# Autodesk Inventor assembly: printer2
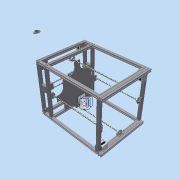
[picture p0: Inventor's stored thumbnail of the model, 180x180]
Saved by Autodesk Inventor 2015 (Build 190159000, 159)
## iProperties
Created: 2016-06-24
Part Number: printer2
Document SubType Name: Assembly
Designer: Dustin
Author: Dustin
## Documents named in this file (20)
- E:\Documents\3D Printer\Parts\New Printer\printer2.iam
- E:\Documents\3D Printer\Parts\New Printer\20x20x9in.ipt
- E:\Documents\3D Printer\Parts\New Printer\20x20x27cm.ipt
- E:\Documents\3D Printer\Parts\New Printer\20x20x3in.ipt
- E:\Documents\3D Printer\Parts\New Printer\heated bed.ipt
- E:\Documents\3D Printer\Parts\New Printer\NEMA17.ipt
- E:\Documents\3D Printer\Parts\New Printer\.375 - 8 (4 start) acme thread.ipt
- E:\Documents\3D Printer\Parts\New Printer\leadscrew corners.ipt
- E:\Documents\3D Printer\Parts\New Printer\bed plate.ipt
- E:\Documents\3D Printer\Parts\New Printer\Imported Components\GT2_20teeth_pulley\GT2_20teeth_pulley.ipt
- E:\Documents\3D Printer\Parts\New Printer\6mm_rod_265.ipt
- E:\Documents\3D Printer\Parts\New Printer\motor mount.ipt
- E:\Documents\3D Printer\Parts\New Printer\20x20x5cm.ipt
- E:\Documents\3D Printer\Parts\New Printer\extruder.iam
- E:\Documents\3D Printer\Parts\New Printer\X smooth mount.ipt
- E:\Documents\3D Printer\Parts\New Printer\m3x20.ipt
- E:\Documents\3D Printer\Parts\New Printer\Corner mount.ipt
- E:\Documents\3D Printer\Parts\New Printer\m4 bearing assembly.iam
- E:\Documents\3D Printer\Parts\New Printer\m4 bearing assembly 30mm.iam
- E:\Documents\3D Printer\Parts\New Printer\KFL08.iam
## Components (83 placed, 19 different names)
1. 20x20x9in:1 — Mate:2, Flush:3, Flush:4, Flush:7
2. 20x20x9in:2 — Mate:4, Flush:8, Flush:9, Mate:6, Mate:39, Mate:52, Flush:53, Flush:64, Mate:66
3. 20x20x9in:3 — Mate:5, Flush:10, Flush:11, Flush:12, Flush:13, Mate:48, Flush:51, Mate:59, Flush:65, Mate:67
4. 20x20x9in:4 — Mate:1, Flush:1, Flush:2, Mate:3, Flush:5, Flush:6
5. 20x20x27cm:1 — Mate:1, Flush:1, Flush:2, Mate:2, Flush:3, Flush:4, Mate:38, Flush:40, Flush:41
6. 20x20x27cm:2 — Mate:3, Flush:5, Flush:6, Flush:7
7. 20x20x27cm:3 — Mate:4, Flush:8, Flush:9, Mate:5, Flush:10, Flush:11, Mate:11, Mate:12, Flush:24, Flush:25, Flush:26, Flush:27, Mate:50, Mate:60, Flush:60, Flush:61, Mate:65, Mate:85
8. 20x20x27cm:4 — Mate:6, Flush:12, Flush:13, Mate:10, Mate:13, Flush:21, Flush:22, Flush:23, Flush:28, Flush:29, Mate:54, Flush:54, Flush:62, Mate:61, Flush:63, Mate:68
9. 20x20x27cm:5 — Mate:13, Flush:21, Flush:28, Flush:29
10. 20x20x27cm:6 — Mate:12, Flush:26, Flush:27, Mate:14, Flush:30, Flush:31
11. 20x20x27cm:7 — Mate:11, Flush:24, Flush:25
12. 20x20x27cm:8 — Mate:10, Flush:22, Flush:23
13. 20x20x3in:1 — Mate:37, Flush:32, Flush:33
14. 20x20x3in:2 — Mate:36, Flush:38, Flush:39, Mate:38, Flush:40, Flush:41
15. 20x20x3in:3 — Mate:34, Flush:36, Flush:37
16. 20x20x3in:4 — Mate:35, Flush:34, Flush:35
17. 20x20x9in:5 — Mate:40, Flush:47, Flush:48, Flush:73, Flush:105
18. 20x20x9in:6 — Mate:44, Flush:50, Flush:77, Mate:83, Flush:104
19. 20x20x27cm:9 — Mate:14, Flush:30, Flush:31, Mate:34, Mate:37, Flush:32, Flush:33, Flush:38, Flush:39, Mate:42, Flush:49, Mate:74, Mate:75, Flush:74, Flush:75, Flush:76, Angle:3
20. 20x20x27cm:10 — Mate:35, Mate:36, Flush:34, Flush:35, Flush:36, Flush:37, Mate:46, Flush:71, Flush:72, Mate:72, Mate:73, Flush:78
21. heated bed:1 — Mate:58, Tangent:5, Tangent:6
22. NEMA17:1 — Mate:39, Flush:64, Insert:7, Mate:85, Insert:25, Insert:26
23. NEMA17:2 — Mate:59, Flush:65, Insert:6, Insert:20, Insert:21
24. .375 - 8 (4 start) acme thread:1 — Tangent:1, Flush:58, Insert:3, Tangent:18, Tangent:24, Tangent:56
25. .375 - 8 (4 start) acme thread:2 — Tangent:4, Flush:57, Insert:1, Tangent:20, Tangent:25, Tangent:54
26. .375 - 8 (4 start) acme thread:3 — Tangent:3, Flush:56, Insert:5, Tangent:14
27. .375 - 8 (4 start) acme thread:4 — Tangent:2, Flush:55, Insert:4, Tangent:16, Tangent:21, Tangent:53
28. leadscrew corners:1 — Mate:40, Flush:47, Tangent:1, Mate:57, Tangent:57, Flush:111
29. leadscrew corners:2 — Mate:42, Flush:48, Tangent:4, Mate:80, Flush:110, Tangent:55
30. leadscrew corners:3 — Mate:44, Flush:49, Tangent:3
31. leadscrew corners:4 — Mate:46, Flush:50, Tangent:2, Flush:109
32. leadscrew corners:5 — Mate:48, Flush:51, Flush:58, Tangent:18, Mate:67
33. leadscrew corners:6 — Mate:50, Flush:57, Tangent:20, Mate:65
34. leadscrew corners:7 — Mate:54, Flush:54, Flush:55, Tangent:16, Mate:68
35. leadscrew corners:8 — Mate:52, Flush:53, Flush:56, Tangent:14, Mate:66
36. bed plate:1 — Mate:57, Mate:58, Tangent:5, Tangent:6, Mate:80, Tangent:21, Tangent:24, Tangent:25, Angle:3
37. GT2_20teeth_pulley:1 — Insert:1
38. GT2_20teeth_pulley:2 — Insert:5
39. GT2_20teeth_pulley:3 — Insert:3
40. GT2_20teeth_pulley:4 — Insert:4
41. 20x20x27cm:11 — Mate:60, Flush:60, Flush:61
42. 20x20x27cm:12 — Flush:62, Mate:61, Flush:63
43. GT2_20teeth_pulley:5 — Insert:6
44. GT2_20teeth_pulley:6 — Insert:7
45. 6mm_rod_265:1 — Flush:68, Mate:83, Angle:1, Tangent:22, Insert:28, Tangent:47, Insert:33, Tangent:51, Angle:26, Angle:27
46. 6mm_rod_265:2 — Flush:68, Tangent:23, Insert:27, Tangent:48, Angle:25, Tangent:52
47. NEMA17:3 — Insert:18, Insert:19, Mate:87, Mate:88, Insert:32
48. NEMA17:4 — Insert:23, Insert:24, Mate:90, Tangent:34, Insert:31, Mate:98
49. motor mount:1 — Insert:18, Insert:19, Mate:86
50. 20x20x5cm:1 — Flush:71, Flush:72, Mate:72
51. 20x20x5cm:2 — Mate:75, Flush:73, Flush:74
52. 20x20x5cm:3 — Mate:74, Flush:75, Flush:76, Flush:79, Flush:80, Mate:76
53. 20x20x5cm:4 — Mate:73, Flush:77, Flush:78, Mate:77, Flush:81, Flush:82
54. 20x20x27cm:13 — Mate:77, Flush:81, Flush:82, Mate:88, Mate:90
55. 20x20x27cm:14 — Flush:79, Flush:80, Mate:76, Mate:78, Flush:83, Flush:84, Mate:79, Flush:85, Flush:86, Flush:89, Mate:100, Flush:92
56. 20x20x9in:7 — Mate:78, Flush:83, Flush:84, Angle:2, Mate:84, Mate:89, Mate:98, Flush:91, Mate:101, Flush:106
57. 20x20x9in:8 — Mate:79, Flush:85, Flush:86, Mate:86, Mate:87, Flush:90
58. motor mount:2 — Insert:20, Insert:21
59. GT2_20teeth_pulley:7 — Insert:32
60. motor mount:3 — Insert:23, Insert:24, Mate:89
61. extruder:1 [sub-assembly] — Angle:1, Angle:2, Tangent:22, Tangent:23, Mate:84, Tangent:35, Angle:11, Mate:99, Tangent:36, Angle:12, Mate:102, Angle:21, Tangent:45, Angle:22, Tangent:46, Flush:100, Flush:101, Flush:106, Flush:107, Angle:27, Flush:108
62. motor mount:4 — Insert:25, Insert:26
63. X smooth mount:1 — Insert:27, Insert:28, Angle:13, Tangent:37, Flush:93, Angle:16, Tangent:40, Flush:95, Tangent:51, Angle:25, Flush:104, Tangent:52
64. GT2_20teeth_pulley:8 — Tangent:34, Insert:31
65. m3x20:1 — Tangent:35, Angle:11, Mate:99, Flush:107
66. Corner mount:1 — Flush:89, Mate:100, Flush:90, Angle:19, Flush:98, Tangent:43, Angle:20, Tangent:44, Flush:99
67. Corner mount:2 — Flush:91, Mate:101, Flush:92, Angle:14, Tangent:38, Flush:94, Angle:15, Tangent:39, Mate:103
68. m3x20:2 — Tangent:36, Angle:12, Mate:102, Flush:108
69. m4 bearing assembly:1 [sub-assembly] — Angle:13, Tangent:37, Flush:93
70. m4 bearing assembly:2 [sub-assembly] — Angle:14, Tangent:38, Flush:94
71. m4 bearing assembly 30mm:1 [sub-assembly] — Angle:15, Tangent:39, Mate:103
72. m4 bearing assembly 30mm:2 [sub-assembly] — Angle:16, Tangent:40, Flush:95
73. m4 bearing assembly:3 [sub-assembly] — Tangent:50, Angle:24, Flush:103
74. m4 bearing assembly 30mm:3 [sub-assembly] — Tangent:49, Angle:23, Flush:102
75. m4 bearing assembly:4 [sub-assembly] — Angle:19, Flush:98, Tangent:43
76. m4 bearing assembly 30mm:4 [sub-assembly] — Angle:20, Tangent:44, Flush:99
77. m3x20:3 — Angle:21, Tangent:45, Flush:100
78. m3x20:4 — Angle:22, Tangent:46, Flush:101
79. X smooth mount:2 — Tangent:47, Tangent:48, Insert:33, Tangent:49, Tangent:50, Angle:23, Angle:24, Flush:102, Flush:103, Angle:26, Flush:105
80. KFL08:1 [sub-assembly] — Flush:109, Tangent:53
81. KFL08:2 [sub-assembly] — Flush:110, Tangent:54, Tangent:55
82. KFL08:3 [sub-assembly]
83. KFL08:4 [sub-assembly] — Tangent:56, Tangent:57, Flush:111
## Relationships (230: Flush 96, Mate 60, Tangent 37, Insert 19, Angle 18)
- Mate:1: 20x20x9in:4 ↔ 20x20x27cm:1
- Flush:1: 20x20x9in:4 ↔ 20x20x27cm:1
- Flush:2: 20x20x9in:4 ↔ 20x20x27cm:1
- Mate:2: 20x20x9in:1 ↔ 20x20x27cm:1
- Flush:3: 20x20x9in:1 ↔ 20x20x27cm:1
- Flush:4: 20x20x9in:1 ↔ 20x20x27cm:1
- Mate:3: 20x20x9in:4 ↔ 20x20x27cm:2
- Flush:5: 20x20x9in:4 ↔ 20x20x27cm:2
- Flush:6: 20x20x9in:4 ↔ 20x20x27cm:2
- Flush:7: 20x20x9in:1 ↔ 20x20x27cm:2
- Mate:4: 20x20x9in:2 ↔ 20x20x27cm:3
- Flush:8: 20x20x9in:2 ↔ 20x20x27cm:3
- Flush:9: 20x20x9in:2 ↔ 20x20x27cm:3
- Mate:5: 20x20x9in:3 ↔ 20x20x27cm:3
- Flush:10: 20x20x9in:3 ↔ 20x20x27cm:3
- Flush:11: 20x20x9in:3 ↔ 20x20x27cm:3
- Mate:6: 20x20x9in:2 ↔ 20x20x27cm:4
- Flush:12: 20x20x9in:3 ↔ 20x20x27cm:4
- Flush:13: 20x20x9in:3 ↔ 20x20x27cm:4
- [Mate]: 20x20x9in:6 ↔ 20x20x27cm:9
- [Flush]: 20x20x9in:6 ↔ 20x20x27cm:9
- [Flush]: 20x20x9in:6 ↔ 20x20x27cm:9
- [Mate]: 20x20x9in:5 ↔ 20x20x27cm:9
- [Flush]: 20x20x9in:5 ↔ 20x20x27cm:9
- [Flush]: 20x20x9in:5 ↔ 20x20x27cm:9
- [Mate]: 20x20x9in:6 ↔ 20x20x27cm:10
- [Flush]: 20x20x9in:6 ↔ 20x20x27cm:10
- [Flush]: 20x20x9in:6 ↔ 20x20x27cm:10
- [Flush]: 20x20x9in:5 ↔ 20x20x27cm:10
- Mate:10: 20x20x27cm:4 ↔ 20x20x27cm:8
- Mate:11: 20x20x27cm:3 ↔ 20x20x27cm:7
- Mate:12: 20x20x27cm:3 ↔ 20x20x27cm:6
- Mate:13: 20x20x27cm:4 ↔ 20x20x27cm:5
- Flush:21: 20x20x27cm:4 ↔ 20x20x27cm:5
- Flush:22: 20x20x27cm:4 ↔ 20x20x27cm:8
- Flush:23: 20x20x27cm:4 ↔ 20x20x27cm:8
- Flush:24: 20x20x27cm:3 ↔ 20x20x27cm:7
- Flush:25: 20x20x27cm:3 ↔ 20x20x27cm:7
- Flush:26: 20x20x27cm:3 ↔ 20x20x27cm:6
- Flush:27: 20x20x27cm:3 ↔ 20x20x27cm:6
- Flush:28: 20x20x27cm:4 ↔ 20x20x27cm:5
- Flush:29: 20x20x27cm:4 ↔ 20x20x27cm:5
- Mate:14: 20x20x27cm:6 ↔ 20x20x27cm:9
- Flush:30: 20x20x27cm:6 ↔ 20x20x27cm:9
- Flush:31: 20x20x27cm:6 ↔ 20x20x27cm:9
- Mate:35: 20x20x3in:4 ↔ 20x20x27cm:10
- Mate:34: 20x20x3in:3 ↔ 20x20x27cm:9
- Mate:36: 20x20x3in:2 ↔ 20x20x27cm:10
- Mate:37: 20x20x3in:1 ↔ 20x20x27cm:9
- Flush:32: 20x20x3in:1 ↔ 20x20x27cm:9
- Flush:33: 20x20x3in:1 ↔ 20x20x27cm:9
- Flush:34: 20x20x3in:4 ↔ 20x20x27cm:10
- Flush:35: 20x20x3in:4 ↔ 20x20x27cm:10
- Flush:36: 20x20x3in:3 ↔ 20x20x27cm:10
- Flush:37: 20x20x3in:3 ↔ 20x20x27cm:10
- Flush:38: 20x20x3in:2 ↔ 20x20x27cm:9
- Flush:39: 20x20x3in:2 ↔ 20x20x27cm:9
- Mate:38: 20x20x27cm:1 ↔ 20x20x3in:2
- Flush:40: 20x20x27cm:1 ↔ 20x20x3in:2
- Flush:41: 20x20x27cm:1 ↔ 20x20x3in:2
- Mate:39: 20x20x9in:2 ↔ NEMA17:1
- Mate:40: 20x20x9in:5 ↔ leadscrew corners:1
- Flush:47: 20x20x9in:5 ↔ leadscrew corners:1
- Tangent:1: .375 - 8 (4 start) acme thread:1 ↔ leadscrew corners:1
- Mate:42: 20x20x27cm:9 ↔ leadscrew corners:2
- Flush:48: 20x20x9in:5 ↔ leadscrew corners:2
- Mate:44: 20x20x9in:6 ↔ leadscrew corners:3
- Flush:49: 20x20x27cm:9 ↔ leadscrew corners:3
- Mate:46: 20x20x27cm:10 ↔ leadscrew corners:4
- Flush:50: 20x20x9in:6 ↔ leadscrew corners:4
- Tangent:2: .375 - 8 (4 start) acme thread:4 ↔ leadscrew corners:4
- Tangent:3: .375 - 8 (4 start) acme thread:3 ↔ leadscrew corners:3
- Tangent:4: .375 - 8 (4 start) acme thread:2 ↔ leadscrew corners:2
- Mate:48: 20x20x9in:3 ↔ leadscrew corners:5
- Flush:51: 20x20x9in:3 ↔ leadscrew corners:5
- Mate:50: 20x20x27cm:3 ↔ leadscrew corners:6
- Mate:52: 20x20x9in:2 ↔ leadscrew corners:8
- Flush:53: 20x20x9in:2 ↔ leadscrew corners:8
- Mate:54: 20x20x27cm:4 ↔ leadscrew corners:7
- Flush:54: 20x20x27cm:4 ↔ leadscrew corners:7
- Flush:55 (5 mm): .375 - 8 (4 start) acme thread:4 ↔ leadscrew corners:7
- Flush:56 (5 mm): .375 - 8 (4 start) acme thread:3 ↔ leadscrew corners:8
- Flush:57 (5 mm): .375 - 8 (4 start) acme thread:2 ↔ leadscrew corners:6
- Flush:58 (5 mm): .375 - 8 (4 start) acme thread:1 ↔ leadscrew corners:5
- Mate:57: leadscrew corners:1 ↔ bed plate:1
- Mate:58 (6 mm): heated bed:1 ↔ bed plate:1
- Tangent:5: heated bed:1 ↔ bed plate:1
- Tangent:6: heated bed:1 ↔ bed plate:1
- Mate:59: 20x20x9in:3 ↔ NEMA17:2
- Insert:1 (-19.05 mm): .375 - 8 (4 start) acme thread:2 ↔ GT2_20teeth_pulley:1
- Insert:3 (-19.05 mm): .375 - 8 (4 start) acme thread:1 ↔ GT2_20teeth_pulley:3
- Insert:4 (-19.05 mm): .375 - 8 (4 start) acme thread:4 ↔ GT2_20teeth_pulley:4
- Insert:5 (-19.05 mm): .375 - 8 (4 start) acme thread:3 ↔ GT2_20teeth_pulley:2
- Mate:60: 20x20x27cm:3 ↔ 20x20x27cm:11
- Flush:60: 20x20x27cm:3 ↔ 20x20x27cm:11
- Flush:61: 20x20x27cm:3 ↔ 20x20x27cm:11
- Flush:62: 20x20x27cm:4 ↔ 20x20x27cm:12
- Mate:61: 20x20x27cm:4 ↔ 20x20x27cm:12
- Flush:63: 20x20x27cm:4 ↔ 20x20x27cm:12
- Flush:64: 20x20x9in:2 ↔ NEMA17:1
- Flush:65: 20x20x9in:3 ↔ NEMA17:2
- Insert:6 (-3.81 mm): NEMA17:2 ↔ GT2_20teeth_pulley:5
- Insert:7 (-3.81 mm): NEMA17:1 ↔ GT2_20teeth_pulley:6
- Flush:68: 6mm_rod_265:1 ↔ 6mm_rod_265:2
- Tangent:14: .375 - 8 (4 start) acme thread:3 ↔ leadscrew corners:8
- Tangent:16 (-1 mm): .375 - 8 (4 start) acme thread:4 ↔ leadscrew corners:7
- Tangent:18: .375 - 8 (4 start) acme thread:1 ↔ leadscrew corners:5
- Tangent:20 (-1 mm): .375 - 8 (4 start) acme thread:2 ↔ leadscrew corners:6
- Mate:65: 20x20x27cm:3 ↔ leadscrew corners:6
- Mate:66: 20x20x9in:2 ↔ leadscrew corners:8
- Mate:67: 20x20x9in:3 ↔ leadscrew corners:5
- Mate:68: 20x20x27cm:4 ↔ leadscrew corners:7
- Insert:18: NEMA17:3 ↔ motor mount:1
- Insert:19: NEMA17:3 ↔ motor mount:1
- Flush:71: 20x20x27cm:10 ↔ 20x20x5cm:1
- Flush:72: 20x20x27cm:10 ↔ 20x20x5cm:1
- Mate:72: 20x20x27cm:10 ↔ 20x20x5cm:1
- Mate:73: 20x20x27cm:10 ↔ 20x20x5cm:4
- Mate:74: 20x20x27cm:9 ↔ 20x20x5cm:3
- Mate:75: 20x20x27cm:9 ↔ 20x20x5cm:2
- Flush:73: 20x20x9in:5 ↔ 20x20x5cm:2
- Flush:74: 20x20x27cm:9 ↔ 20x20x5cm:2
- Flush:75: 20x20x27cm:9 ↔ 20x20x5cm:3
- Flush:76: 20x20x27cm:9 ↔ 20x20x5cm:3
- Flush:77: 20x20x9in:6 ↔ 20x20x5cm:4
- Flush:78: 20x20x27cm:10 ↔ 20x20x5cm:4
- Flush:79: 20x20x5cm:3 ↔ 20x20x27cm:14
- Flush:80: 20x20x5cm:3 ↔ 20x20x27cm:14
- Mate:76: 20x20x5cm:3 ↔ 20x20x27cm:14
- Mate:77: 20x20x5cm:4 ↔ 20x20x27cm:13
- Flush:81: 20x20x5cm:4 ↔ 20x20x27cm:13
- Flush:82: 20x20x5cm:4 ↔ 20x20x27cm:13
- Mate:78: 20x20x27cm:14 ↔ 20x20x9in:7
- Flush:83: 20x20x27cm:14 ↔ 20x20x9in:7
- Flush:84: 20x20x27cm:14 ↔ 20x20x9in:7
- Mate:79: 20x20x27cm:14 ↔ 20x20x9in:8
- Flush:85: 20x20x27cm:14 ↔ 20x20x9in:8
- Flush:86: 20x20x27cm:14 ↔ 20x20x9in:8
- Insert:20: NEMA17:2 ↔ motor mount:2
- Insert:21: NEMA17:2 ↔ motor mount:2
- Mate:80: leadscrew corners:2 ↔ bed plate:1
- Tangent:21: .375 - 8 (4 start) acme thread:4 ↔ bed plate:1
- Insert:23: NEMA17:4 ↔ motor mount:3
- Insert:24: NEMA17:4 ↔ motor mount:3
- Mate:83: 20x20x9in:6 ↔ 6mm_rod_265:1
- Angle:1 (0 deg): 6mm_rod_265:1 ↔ extruder:1
- Angle:2 (180 deg): 20x20x9in:7 ↔ extruder:1
- Tangent:22: 6mm_rod_265:1 ↔ extruder:1
- Tangent:23: 6mm_rod_265:2 ↔ extruder:1
- Mate:84 (25 mm): 20x20x9in:7 ↔ extruder:1
- Mate:85: 20x20x27cm:3 ↔ NEMA17:1
- Insert:25: NEMA17:1 ↔ motor mount:4
- Insert:26: NEMA17:1 ↔ motor mount:4
- Insert:27: 6mm_rod_265:2 ↔ X smooth mount:1
- Insert:28: 6mm_rod_265:1 ↔ X smooth mount:1
- Tangent:24: .375 - 8 (4 start) acme thread:1 ↔ bed plate:1
- Tangent:25: .375 - 8 (4 start) acme thread:2 ↔ bed plate:1
- Angle:3 (0 deg): 20x20x27cm:9 ↔ bed plate:1
- Mate:86: motor mount:1 ↔ 20x20x9in:8
- Mate:87: NEMA17:3 ↔ 20x20x9in:8
- Mate:88: NEMA17:3 ↔ 20x20x27cm:13
- Mate:89: 20x20x9in:7 ↔ motor mount:3
- Mate:90: NEMA17:4 ↔ 20x20x27cm:13
- Tangent:34: NEMA17:4 ↔ GT2_20teeth_pulley:8
- Insert:31 (5 mm): NEMA17:4 ↔ GT2_20teeth_pulley:8
- Mate:98: NEMA17:4 ↔ 20x20x9in:7
- Tangent:35: extruder:1 ↔ m3x20:1
- Angle:11 (180 deg): extruder:1 ↔ m3x20:1
- Mate:99 (14 mm): extruder:1 ↔ m3x20:1
- Flush:89: 20x20x27cm:14 ↔ Corner mount:1
- Mate:100: 20x20x27cm:14 ↔ Corner mount:1
- Flush:90: 20x20x9in:8 ↔ Corner mount:1
- Flush:91: 20x20x9in:7 ↔ Corner mount:2
- Mate:101: 20x20x9in:7 ↔ Corner mount:2
- Flush:92: 20x20x27cm:14 ↔ Corner mount:2
- Insert:32: NEMA17:3 ↔ GT2_20teeth_pulley:7
- Tangent:36: extruder:1 ↔ m3x20:2
- Angle:12 (180 deg): extruder:1 ↔ m3x20:2
- Mate:102 (10 mm): extruder:1 ↔ m3x20:2
- Angle:13 (180 deg): X smooth mount:1 ↔ m4 bearing assembly:1
- Tangent:37: X smooth mount:1 ↔ m4 bearing assembly:1
- Flush:93 (-5 mm): X smooth mount:1 ↔ m4 bearing assembly:1
- Angle:14 (0 deg): Corner mount:2 ↔ m4 bearing assembly:2
- Tangent:38: Corner mount:2 ↔ m4 bearing assembly:2
- Flush:94 (-6 mm): Corner mount:2 ↔ m4 bearing assembly:2
- Angle:15 (0 deg): Corner mount:2 ↔ m4 bearing assembly 30mm:1
- Tangent:39: Corner mount:2 ↔ m4 bearing assembly 30mm:1
- Mate:103 (15 mm): Corner mount:2 ↔ m4 bearing assembly 30mm:1
- Angle:16 (180 deg): X smooth mount:1 ↔ m4 bearing assembly 30mm:2
- Tangent:40: X smooth mount:1 ↔ m4 bearing assembly 30mm:2
- Flush:95: X smooth mount:1 ↔ m4 bearing assembly 30mm:2
- Angle:19 (0 deg): Corner mount:1 ↔ m4 bearing assembly:4
- Flush:98 (-6 mm): Corner mount:1 ↔ m4 bearing assembly:4
- Tangent:43: Corner mount:1 ↔ m4 bearing assembly:4
- Angle:20 (180 deg): Corner mount:1 ↔ m4 bearing assembly 30mm:4
- Tangent:44: Corner mount:1 ↔ m4 bearing assembly 30mm:4
- Flush:99 (1 mm): Corner mount:1 ↔ m4 bearing assembly 30mm:4
- Angle:21 (180 deg): extruder:1 ↔ m3x20:3
- Tangent:45: extruder:1 ↔ m3x20:3
- Angle:22 (180 deg): extruder:1 ↔ m3x20:4
- Tangent:46: extruder:1 ↔ m3x20:4
- Flush:100 (-6 mm): extruder:1 ↔ m3x20:3
- Flush:101 (-2 mm): extruder:1 ↔ m3x20:4
- Tangent:47: 6mm_rod_265:1 ↔ X smooth mount:2
- Tangent:48: 6mm_rod_265:2 ↔ X smooth mount:2
- Insert:33 (-20 mm): 6mm_rod_265:1 ↔ X smooth mount:2
- Tangent:49: m4 bearing assembly 30mm:3 ↔ X smooth mount:2
- Tangent:50: m4 bearing assembly:3 ↔ X smooth mount:2
- Angle:23 (180 deg): m4 bearing assembly 30mm:3 ↔ X smooth mount:2
- Angle:24 (180 deg): m4 bearing assembly:3 ↔ X smooth mount:2
- Flush:102: m4 bearing assembly 30mm:3 ↔ X smooth mount:2
- Flush:103 (-5 mm): m4 bearing assembly:3 ↔ X smooth mount:2
- Tangent:51: 6mm_rod_265:1 ↔ X smooth mount:1
- Angle:25 (0 deg): 6mm_rod_265:2 ↔ X smooth mount:1
- Flush:104: 20x20x9in:6 ↔ X smooth mount:1
- Tangent:52: 6mm_rod_265:2 ↔ X smooth mount:1
- Angle:26 (0 deg): 6mm_rod_265:1 ↔ X smooth mount:2
- Flush:105: 20x20x9in:5 ↔ X smooth mount:2
- Flush:106 (47 mm): 20x20x9in:7 ↔ extruder:1
- Flush:107: extruder:1 ↔ m3x20:1
- Angle:27 (0 deg): 6mm_rod_265:1 ↔ extruder:1
- Flush:108 (-5 mm): extruder:1 ↔ m3x20:2
- Flush:109: leadscrew corners:4 ↔ KFL08:1
- Tangent:53: .375 - 8 (4 start) acme thread:4 ↔ KFL08:1
- Flush:110: leadscrew corners:2 ↔ KFL08:2
- Tangent:54: .375 - 8 (4 start) acme thread:2 ↔ KFL08:2
- Tangent:55: leadscrew corners:2 ↔ KFL08:2
- Tangent:56: .375 - 8 (4 start) acme thread:1 ↔ KFL08:4
- Tangent:57: leadscrew corners:1 ↔ KFL08:4
- Flush:111: leadscrew corners:1 ↔ KFL08:4
## Named parameters: d25_d15 = 0 mm, d26_d6 = 0 mm, d27_d7 = 0 mm, d28_d8 = 0 mm, d29_d9 = 0 mm, d30_d10 = 0 mm, d31_d11 = 0 mm, d32_d12 = 0 mm, d33_d13 = 0 mm, d34_d14 = 0 mm
